# Autodesk Inventor assembly: 000 ASY GBK Gubkinskiy
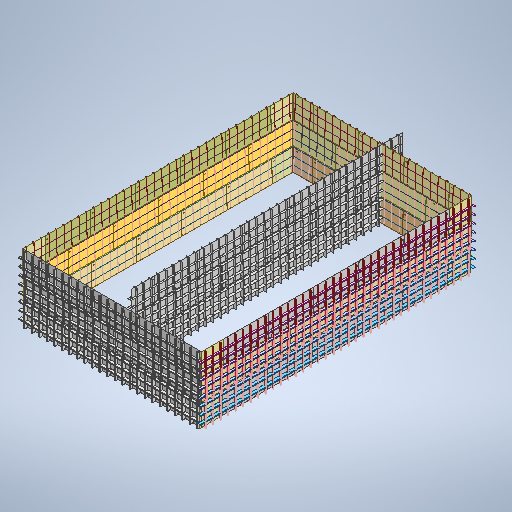
[picture p0: Inventor's stored thumbnail of the model, 512x512]
Saved by Autodesk Inventor 2026 (Build 300175000, 175)
## iProperties
Created: 2026-04-17
Part Number: 000 ASY GBK Gubkinskiy
Document SubType Name: Assembly
Designer: admin
Mass: 2.0116e+07 g
Surface Area: 1.3016e+07 cm^2
Volume: 2.56254e+06 cm^3
Density: 7.85 g/cm^3
Author: admin
## Documents named in this file (6)
- C:\Users\pokla\Documents\Inventor\GBK-Gubkinskiy\000 ASY GBK Gubkinskiy.iam
- C:\Users\pokla\Documents\Inventor\GBK-Gubkinskiy\GBK bottom.ipt
- C:\Users\pokla\Documents\Inventor\GBK-Gubkinskiy\ASY GBK длинная стенка.iam
- C:\Users\pokla\Documents\Inventor\GBK-Gubkinskiy\090 ASY bottom.iam
- C:\Users\pokla\Documents\Inventor\GBK-Gubkinskiy\ASY GBK короткая стенка.iam
- C:\Users\pokla\Documents\Inventor\GBK-Gubkinskiy\ASY GBK центральная стенка.iam
## Components (7 placed, 5 different names)
1. GBK bottom.ipt:1 — Заподлицо:8, Заподлицо:9, Совмещение:20, Совмещение:21, Заподлицо:14, Заподлицо:15, Совмещение:22, Заподлицо:16, Совмещение:23, Заподлицо:19, Заподлицо:20, Заподлицо:21, Заподлицо:22, Совмещение:24, Совмещение:25, Совмещение:26
2. ASY GBK длинная стенка.iam:1 [sub-assembly] — Заподлицо:15, Заподлицо:20
3. ASY GBK длинная стенка.iam:2 [sub-assembly] — Заподлицо:9, Совмещение:21, Заподлицо:14
4. 090 ASY bottom.iam:1 [sub-assembly] — Совмещение:19, Заподлицо:8
5. ASY GBK короткая стенка.iam:1 [sub-assembly] — Совмещение:20, Заподлицо:19, Совмещение:25
6. ASY GBK короткая стенка.iam:2 [sub-assembly] — Совмещение:22, Заподлицо:16, Совмещение:26
7. ASY GBK центральная стенка.iam:1 [sub-assembly] — Совмещение:23, Заподлицо:18
## Relationships (19: Flush 10, Mate 9)
- [Mate]: GBK bottom.ipt:1 ↔ ASY GBK длинная стенка.iam:1
- Совмещение:19 [Mate]: 090 ASY bottom.iam:1
- Заподлицо:8 [Flush]: GBK bottom.ipt:1 ↔ 090 ASY bottom.iam:1
- Заподлицо:9 [Flush] (-120 mm): GBK bottom.ipt:1 ↔ ASY GBK длинная стенка.iam:2
- Совмещение:20 [Mate]: GBK bottom.ipt:1 ↔ ASY GBK короткая стенка.iam:1
- Совмещение:21 [Mate]: GBK bottom.ipt:1 ↔ ASY GBK длинная стенка.iam:2
- Заподлицо:14 [Flush] (40 mm): GBK bottom.ipt:1 ↔ ASY GBK длинная стенка.iam:2
- Заподлицо:15 [Flush] (40 mm): GBK bottom.ipt:1 ↔ ASY GBK длинная стенка.iam:1
- Совмещение:22 [Mate]: GBK bottom.ipt:1 ↔ ASY GBK короткая стенка.iam:2
- Заподлицо:16 [Flush] (40 mm): GBK bottom.ipt:1 ↔ ASY GBK короткая стенка.iam:2
- Совмещение:23 [Mate]: GBK bottom.ipt:1 ↔ ASY GBK центральная стенка.iam:1
- Заподлицо:18 [Flush] (-2 mm): ASY GBK центральная стенка.iam:1
- Заподлицо:19 [Flush] (40 mm): GBK bottom.ipt:1 ↔ ASY GBK короткая стенка.iam:1
- Заподлицо:20 [Flush] (120 mm): GBK bottom.ipt:1 ↔ ASY GBK длинная стенка.iam:1
- Заподлицо:21 [Flush]: GBK bottom.ipt:1
- Заподлицо:22 [Flush]: GBK bottom.ipt:1
- Совмещение:24 [Mate]: GBK bottom.ipt:1
- Совмещение:25 [Mate] (-360 mm): GBK bottom.ipt:1 ↔ ASY GBK короткая стенка.iam:1
- Совмещение:26 [Mate] (-360 mm): GBK bottom.ipt:1 ↔ ASY GBK короткая стенка.iam:2
## Named parameters: Зазор_по_горизонту = 1 mm, d120_Зазор_по_горизонту = 1 mm, d141_Зазор_по_горизонту = 1 mm, d159_d141_Зазор_по_горизонту = 1 mm, d175_d141_Зазор_по_горизонту = 1 mm
